# Autodesk Inventor assembly: WheelsScoringPlatform
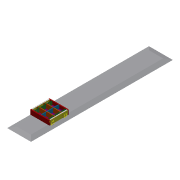
[picture p0: Inventor's stored thumbnail of the model, 180x180]
Saved by Autodesk Inventor 2015 (Build 190159000, 159)
## iProperties
Created: 2015-01-10
Part Number: WheelsScoringPlatform
Document SubType Name: Assembly
Designer: Peter
Author: Peter
## Documents named in this file (4)
- T:\FILES\2015 First Team 1719 CAD Team\2015 Sketches\Strafing the Scoring Platform\WheelsScoringPlatform.iam
- T:\FILES\2015 First Team 1719 CAD Team\2015 Sketches\Strafing the Scoring Platform\Scoring Platform - Lofted Solid Part.ipt
- T:\FILES\2015 First Team 1719 CAD Team\2015 Robot\Chassis, Wheels, and Drive Train\Mechanum Wheel\Chassis - Wheel.iam
- T:\FILES\2015 First Team 1719 CAD Team\2015 Robot\Chassis, Wheels, and Drive Train\Chassis\Full chassis-3.iam
## Components (6 placed, 3 different names)
1. Scoring Platform - Lofted Solid Part:2 — Flush:1, Mate:9
2. Chassis - Wheel:1 [sub-assembly] — Mate:1, Mate:2
3. Chassis - Wheel:2 [sub-assembly] — Mate:7, Mate:8
4. Chassis - Wheel:3 [sub-assembly] — Mate:5, Mate:6
5. Chassis - Wheel:4 [sub-assembly] — Mate:3, Mate:4
6. Full chassis-3:1 [sub-assembly] — Mate:1, Mate:2, Mate:3, Mate:4, Mate:5, Mate:6, Mate:7, Mate:8, Flush:1, Mate:9
## Relationships (10: Mate 9, Flush 1)
- Mate:1: Chassis - Wheel:1 ↔ Full chassis-3:1
- Mate:2 (3.175 mm): Chassis - Wheel:1 ↔ Full chassis-3:1
- Mate:3 (3.175 mm): Chassis - Wheel:4 ↔ Full chassis-3:1
- Mate:4: Chassis - Wheel:4 ↔ Full chassis-3:1
- Mate:5 (3.175 mm): Chassis - Wheel:3 ↔ Full chassis-3:1
- Mate:6: Chassis - Wheel:3 ↔ Full chassis-3:1
- Mate:7: Chassis - Wheel:2 ↔ Full chassis-3:1
- Mate:8: Chassis - Wheel:2 ↔ Full chassis-3:1
- Flush:1: Scoring Platform - Lofted Solid Part:2 ↔ Full chassis-3:1
- Mate:9 (41.148 mm): Scoring Platform - Lofted Solid Part:2 ↔ Full chassis-3:1
